# Autodesk Inventor assembly: 足回り
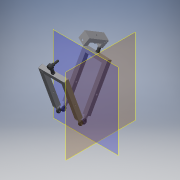
[picture p0: Inventor's stored thumbnail of the model, 180x180]
Saved by Autodesk Inventor 2018 (Build 220112000, 112)
## iProperties
Created: 2017-09-10
Part Number: 足回り
Material: 一般
Document SubType Name: Assembly
Designer: mura5
Author: mura5
## Documents named in this file (3)
- C:\Users\mura5\Documents\RBBR\cart\足回り.iam
- C:\Users\mura5\Documents\RBBR\cart\A.iam
- C:\Users\mura5\Documents\RBBR\cart\車輪取り付け部.iam
## Components (3 placed, 2 different names)
1. A:1 [sub-assembly] — 回転:1
2. A:2 [sub-assembly]
3. 車輪取り付け部:1 [sub-assembly] — 回転:1
## Relationships (1: RevoluteJoint 1)
- 回転:1 [RevoluteJoint]: A:1 ↔ 車輪取り付け部:1
